# Autodesk Inventor assembly: FRAME - OPEN
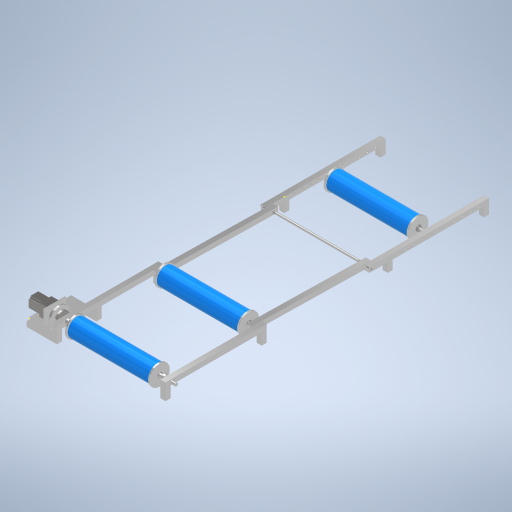
[picture p0: Inventor's stored thumbnail of the model, 512x512]
Saved by Autodesk Inventor 2023 (Build 270158000, 158)
## iProperties
Created: 2022-08-29
Part Number: FRAME - OPEN
Document SubType Name: Assembly
Designer: D.C. Eksteen
Mass: 8630.36 g
Surface Area: 16111.5 cm^2
Volume: 4012.07 cm^3
Density: 2.1511 g/cm^3
Author: D.C. Eksteen
## Documents named in this file (5)
- C:\Users\dylan\Desktop\Skripsie-2022\Design\CAD\FRAME - OPEN.iam
- C:\Users\dylan\Desktop\Skripsie-2022\Design\CAD\REAR ASSEMBLY.iam
- C:\Users\dylan\Desktop\Skripsie-2022\Design\CAD\MIDDLE FRAME.ipt
- C:\Users\dylan\Desktop\Skripsie-2022\Design\CAD\IDLE ROLLER.iam
- C:\Users\dylan\Desktop\Skripsie-2022\Design\CAD\FRONT FRAME ASSEMBLY.iam
## Components (5 placed, 4 different names)
1. FRONT FRAME ASSEMBLY:1 [sub-assembly] — Flush:1
2. REAR ASSEMBLY:1 [sub-assembly] — Mate:3, Mate:4, Mate:5, Mate:6, Flush:1
3. MIDDLE FRAME:1 — Mate:5, Mate:6
4. MIDDLE FRAME:2 — Mate:3, Mate:4
5. IDLE ROLLER:1 [sub-assembly]
## Relationships (11: Mate 9, Angle 1, Flush 1)
- [Mate]: FRONT FRAME ASSEMBLY:1 ↔ MIDDLE FRAME:2
- [Mate] (1 mm): FRONT FRAME ASSEMBLY:1 ↔ MIDDLE FRAME:2
- Mate:3: REAR ASSEMBLY:1 ↔ MIDDLE FRAME:2
- Mate:4 (1 mm): REAR ASSEMBLY:1 ↔ MIDDLE FRAME:2
- [Angle] (0 deg): FRONT FRAME ASSEMBLY:1 ↔ REAR ASSEMBLY:1
- Mate:5: REAR ASSEMBLY:1 ↔ MIDDLE FRAME:1
- Mate:6 (1 mm): REAR ASSEMBLY:1 ↔ MIDDLE FRAME:1
- [Mate]: FRONT FRAME ASSEMBLY:1 ↔ IDLE ROLLER:1
- [Mate]: FRONT FRAME ASSEMBLY:1 ↔ IDLE ROLLER:1
- [Mate]: FRONT FRAME ASSEMBLY:1 ↔ MIDDLE FRAME:1
- Flush:1: FRONT FRAME ASSEMBLY:1 ↔ REAR ASSEMBLY:1
